# Autodesk Inventor assembly: Assembly
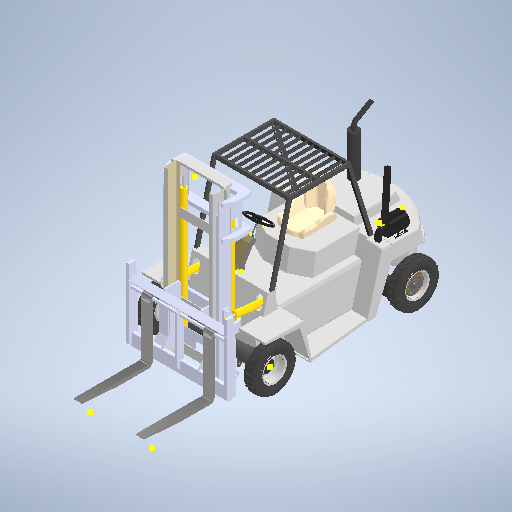
[picture p0: Inventor's stored thumbnail of the model, 512x512]
Saved by Autodesk Inventor 2025 (Build 290162000, 162)
## iProperties
Created: 2024-11-07
Part Number: Assembly
Document SubType Name: Assembly
Designer: SANDHYA
Author: SANDHYA
## Documents named in this file (19)
- C:\Users\ASUS\Downloads\EG parts and assembly\Assembly.iam
- C:\Users\ASUS\Downloads\EG parts and assembly\Prince_ParthP_ParthR_MainBody.ipt
- C:\Users\ASUS\Downloads\EG parts and assembly\Nachiket_Seat.ipt
- C:\Users\ASUS\Downloads\EG parts and assembly\Arjun_RearLight.ipt
- C:\Users\ASUS\Downloads\EG parts and assembly\Devarsh_SteeringWheel.ipt
- C:\Users\ASUS\Downloads\EG parts and assembly\Arjun_SteeringRod.ipt
- C:\Users\ASUS\Downloads\EG parts and assembly\ParthS_HubLink.ipt
- C:\Users\ASUS\Downloads\EG parts and assembly\ParthS_Hub.ipt
- C:\Users\ASUS\Downloads\EG parts and assembly\ParthS_Tyre.ipt
- C:\Users\ASUS\Downloads\EG parts and assembly\Fiza_WheelRim.ipt
- C:\Users\ASUS\Downloads\EG parts and assembly\ParthK_Cylinder1.ipt
- C:\Users\ASUS\Downloads\EG parts and assembly\ParthK_Pushrod1.ipt
- C:\Users\ASUS\Downloads\EG parts and assembly\Parshva_Frame1.ipt
- C:\Users\ASUS\Downloads\EG parts and assembly\Devarsh_AirIntake.ipt
- C:\Users\ASUS\Downloads\EG parts and assembly\ParthK_Frame2.ipt
- C:\Users\ASUS\Downloads\EG parts and assembly\Fiza_Frame3.ipt
- C:\Users\ASUS\Downloads\EG parts and assembly\Arjun_Fork.ipt
- C:\Users\ASUS\Downloads\EG parts and assembly\ParthK_Cylinder2.ipt
- C:\Users\ASUS\Downloads\EG parts and assembly\ParthK_Pushrod2.ipt
## Components (32 placed, 16 different names)
1. Prince_ParthP_ParthR_MainBody:1 — Mate:1, Mate:2, Mate:3, Mate:4, Insert:1, Insert:11, Insert:14, Insert:16, Insert:17, Angle:1, Angle:2, Angle:3, Mate:8, Angle:4, Angle:5, Angle:6
2. Nachiket_Seat:1 — Mate:1
3. Arjun_RearLight:1 — Mate:2
4. Arjun_RearLight:2 — Mate:3
5. Devarsh_SteeringWheel:1 — Mate:4
6. Arjun_SteeringRod:1 — Insert:1, Insert:4, Insert:5
7. ParthS_HubLink:3 — Insert:4, Insert:7
8. ParthS_HubLink:4 — Insert:5, Insert:6
9. ParthS_Hub:3 — Insert:6, Insert:9
10. ParthS_Hub:4 — Insert:7, Insert:15
11. ParthS_Tyre:1 — Insert:12, Insert:14
12. ParthS_Tyre:2 — Insert:10
13. ParthS_Tyre:3 — Insert:13, Insert:15
14. ParthS_Tyre:4 — Insert:8, Insert:9
15. Fiza_WheelRim:1 — Insert:12
16. Fiza_WheelRim:2 — Insert:8
17. Fiza_WheelRim:3 — Insert:13
18. Fiza_WheelRim:4 — Insert:10, Insert:11
19. Parth_Cylinder1:1 — Insert:17, Mate:5
20. Parth_Cylinder1:2 — Insert:16, Mate:6
21. Paerth_Pushrod:1 — Angle:2, Mate:6, Insert:18
22. Paerth_Pushrod:2 — Angle:1, Mate:5, Mate:7
23. Parshva_Frame1:1 — Insert:18, Angle:3, Mate:7, Mate:9, Mate:10, Insert:21, Angle:7, Insert:22, Angle:8, Angle:9, Angle:10
24. Devarsh_AirIntake:1 — Mate:8, Angle:4
25. Parth_Frame2:1 — Mate:9, Mate:10, Mate:11, Mate:12, Mate:15, Mate:16
26. Fiza_Frame3:1 — Mate:11, Mate:12, Insert:19, Insert:20
27. Arjun_Fork:1 — Insert:19, Angle:5
28. Arjun_Fork:2 — Insert:20, Angle:6
29. Parth_Cylinder1:3 — Insert:21, Angle:7, Mate:14
30. Parth_Cylinder1:4 — Insert:22, Angle:8, Mate:13
31. Paerth_Pushrod:3 — Angle:9, Mate:14, Mate:15
32. Paerth_Pushrod:4 — Angle:10, Mate:13, Mate:16
## Relationships (46: Insert 20, Mate 16, Angle 10)
- Mate:1: Prince_ParthP_ParthR_MainBody:1 ↔ Nachiket_Seat:1
- Mate:2: Prince_ParthP_ParthR_MainBody:1 ↔ Arjun_RearLight:1
- Mate:3: Prince_ParthP_ParthR_MainBody:1 ↔ Arjun_RearLight:2
- Mate:4: Prince_ParthP_ParthR_MainBody:1 ↔ Devarsh_SteeringWheel:1
- Insert:1 (20.32 mm): Prince_ParthP_ParthR_MainBody:1 ↔ Arjun_SteeringRod:1
- Insert:4 (-35.56 mm): Arjun_SteeringRod:1 ↔ ParthS_HubLink:3
- Insert:5 (-15.24 mm): Arjun_SteeringRod:1 ↔ ParthS_HubLink:4
- Insert:6 (25.4 mm): ParthS_HubLink:4 ↔ ParthS_Hub:3
- Insert:7 (19.05 mm): ParthS_HubLink:3 ↔ ParthS_Hub:4
- Insert:8 (12.7 mm): ParthS_Tyre:4 ↔ Fiza_WheelRim:2
- Insert:9 (44.45 mm): ParthS_Hub:3 ↔ ParthS_Tyre:4
- Insert:10: ParthS_Tyre:2 ↔ Fiza_WheelRim:4
- Insert:11 (-12.7 mm): Prince_ParthP_ParthR_MainBody:1 ↔ Fiza_WheelRim:4
- Insert:12 (12.7 mm): ParthS_Tyre:1 ↔ Fiza_WheelRim:1
- Insert:13 (-12.7 mm): ParthS_Tyre:3 ↔ Fiza_WheelRim:3
- Insert:14: Prince_ParthP_ParthR_MainBody:1 ↔ ParthS_Tyre:1
- Insert:15 (63.5 mm): ParthS_Hub:4 ↔ ParthS_Tyre:3
- Insert:16 (-31.75 mm): Prince_ParthP_ParthR_MainBody:1 ↔ Parth_Cylinder1:2
- Insert:17 (-31.75 mm): Prince_ParthP_ParthR_MainBody:1 ↔ Parth_Cylinder1:1
- Angle:1 (0 deg): Prince_ParthP_ParthR_MainBody:1 ↔ Paerth_Pushrod:2
- Mate:5: Parth_Cylinder1:1 ↔ Paerth_Pushrod:2
- Angle:2 (0 deg): Prince_ParthP_ParthR_MainBody:1 ↔ Paerth_Pushrod:1
- Mate:6: Parth_Cylinder1:2 ↔ Paerth_Pushrod:1
- Insert:18: Paerth_Pushrod:1 ↔ Parshva_Frame1:1
- Angle:3 (0 deg): Prince_ParthP_ParthR_MainBody:1 ↔ Parshva_Frame1:1
- Mate:7: Paerth_Pushrod:2 ↔ Parshva_Frame1:1
- Mate:8: Prince_ParthP_ParthR_MainBody:1 ↔ Devarsh_AirIntake:1
- Angle:4 (0 deg): Prince_ParthP_ParthR_MainBody:1 ↔ Devarsh_AirIntake:1
- Mate:9 (55 mm): Parshva_Frame1:1 ↔ Parth_Frame2:1
- Mate:10 (37.5 mm): Parshva_Frame1:1 ↔ Parth_Frame2:1
- Mate:11: Parth_Frame2:1 ↔ Fiza_Frame3:1
- Mate:12 (90 mm): Parth_Frame2:1 ↔ Fiza_Frame3:1
- Insert:19 (200 mm): Fiza_Frame3:1 ↔ Arjun_Fork:1
- Insert:20 (200 mm): Fiza_Frame3:1 ↔ Arjun_Fork:2
- Angle:5 (0 deg): Prince_ParthP_ParthR_MainBody:1 ↔ Arjun_Fork:1
- Angle:6 (0 deg): Prince_ParthP_ParthR_MainBody:1 ↔ Arjun_Fork:2
- Insert:21: Parshva_Frame1:1 ↔ Parth_Cylinder1:3
- Angle:7 (180 deg): Parshva_Frame1:1 ↔ Parth_Cylinder1:3
- Insert:22: Parshva_Frame1:1 ↔ Parth_Cylinder1:4
- Angle:8 (180 deg): Parshva_Frame1:1 ↔ Parth_Cylinder1:4
- Angle:9 (0 deg): Parshva_Frame1:1 ↔ Paerth_Pushrod:3
- Angle:10 (0 deg): Parshva_Frame1:1 ↔ Paerth_Pushrod:4
- Mate:13: Parth_Cylinder1:4 ↔ Paerth_Pushrod:4
- Mate:14: Parth_Cylinder1:3 ↔ Paerth_Pushrod:3
- Mate:15: Parth_Frame2:1 ↔ Paerth_Pushrod:3
- Mate:16: Parth_Frame2:1 ↔ Paerth_Pushrod:4
